# Autodesk Inventor assembly: eje
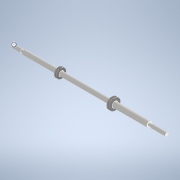
[picture p0: Inventor's stored thumbnail of the model, 180x180]
Saved by Autodesk Inventor 2020 (Build 240168000, 168)
## iProperties
Created: 2021-01-12
Part Number: eje
Document SubType Name: Assembly
Designer: User
Author: User
## Documents named in this file (6)
- D:\Bryan\ESPOL\2020- 2T\Diseño y Simulación de Máquinas\Proyecto2\proyecto2\eje.iam
- D:\Bryan\ESPOL\2020- 2T\Diseño y Simulación de Máquinas\Proyecto2\proyecto2\Eje1.ipt
- D:\Bryan\ESPOL\2020- 2T\Diseño y Simulación de Máquinas\Proyecto2\proyecto2\eje\Design Accelerator\Rodamiento1.iam
- D:\Bryan\ESPOL\2020- 2T\Diseño y Simulación de Máquinas\Proyecto2\proyecto2\eje\Design Accelerator\Rodamiento2.iam
- D:\Bryan\ESPOL\2020- 2T\Diseño y Simulación de Máquinas\Proyecto2\proyecto2\eje\Design Accelerator\Límites y ajustes1.iam
- D:\Bryan\ESPOL\2020- 2T\Diseño y Simulación de Máquinas\Proyecto2\proyecto2\eje\Design Accelerator\Límites y ajustes2.iam
## Components (5 placed, 3 different names)
1. Eje:1 — Coincidencia:1, Coincidencia:2, Coincidencia:3, Coincidencia:4
2. Rodamiento:1 [sub-assembly] — Coincidencia:1, Coincidencia:2
3. Rodamiento:2 [sub-assembly] — Coincidencia:3, Coincidencia:4
4. Límites y ajustes:1 [sub-assembly]
5. Límites y ajustes:2 [sub-assembly]
## Relationships (4: Mate 4)
- Coincidencia:1 [Mate]: Eje:1 ↔ Rodamiento:1
- Coincidencia:2 [Mate]: Eje:1 ↔ Rodamiento:1
- Coincidencia:3 [Mate]: Eje:1 ↔ Rodamiento:2
- Coincidencia:4 [Mate]: Eje:1 ↔ Rodamiento:2
